# Autodesk Inventor assembly: PSU Case
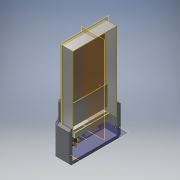
[picture p0: Inventor's stored thumbnail of the model, 180x180]
Saved by Autodesk Inventor 2018 (Build 220112000, 112)
## iProperties
Created: 2018-05-25
Part Number: PSU Case
Document SubType Name: Assembly
Designer: Jasper
Author: Jasper
## Documents named in this file (5)
- C:\Users\Jasper\Downloads\git_WSL\MEME_MACHINE\CAD\PSU Case\PSU Case.iam
- C:\Users\Jasper\Downloads\git_WSL\MEME_MACHINE\CAD\Vitamins\C14 Connector.ipt
- C:\Users\Jasper\Downloads\git_WSL\MEME_MACHINE\CAD\Vitamins\PSU.ipt
- C:\Users\Jasper\Downloads\git_WSL\MEME_MACHINE\CAD\Vitamins\Switch.ipt
- C:\Users\Jasper\Downloads\git_WSL\MEME_MACHINE\CAD\PSU Case\Case.ipt
## Components (4 placed, 4 different names)
1. C14 Connector:1 — Flush:4, Mate:3, Angle:1, Angle:2, Symmetry:1, Mate:4
2. PSU:1 — Mate:2, Mate:3, Angle:1, Angle:2, Flush:5
3. Switch:1 — Mate:2, Flush:4, Symmetry:1, Mate:4, Mate:5
4. Case:1 — Flush:5, Mate:5
## Relationships (9: Mate 4, Flush 2, Angle 2, Symmetry 1)
- Mate:2 (-7.05 mm): PSU:1 ↔ Switch:1
- Flush:4: C14 Connector:1 ↔ Switch:1
- Mate:3: C14 Connector:1 ↔ PSU:1
- Angle:1 (180 deg): C14 Connector:1 ↔ PSU:1
- Angle:2 (180 deg): C14 Connector:1 ↔ PSU:1
- Symmetry:1: C14 Connector:1 ↔ Switch:1
- Mate:4 (25 mm): C14 Connector:1 ↔ Switch:1
- Flush:5: PSU:1 ↔ Case:1
- Mate:5: Switch:1 ↔ Case:1
